# Autodesk Inventor assembly: winch prototype
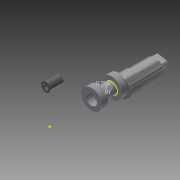
[picture p0: Inventor's stored thumbnail of the model, 180x180]
Saved by Autodesk Inventor 2013 (Build 170138000, 138)
## iProperties
Created: 2013-12-07
Part Number: winch prototype
Document SubType Name: Assembly
Designer: kahohbein
Author: kahohbein
## Documents named in this file (5)
- C:\Users\kahohbein\Documents\GitHub\2013-2014_BlockParty\CAD\Lift\MK2\winch prototype.iam
- C:\Users\kahohbein\Documents\GitHub\2013-2014_BlockParty\CAD\COTSParts\Tetrix\Tetrix hub - motor.ipt
- C:\Users\kahohbein\Documents\GitHub\2013-2014_BlockParty\CAD\COTSParts\Tetrix\Tetrix motor.ipt
- C:\Users\kahohbein\Documents\GitHub\2013-2014_BlockParty\CAD\Lift\MK2\winch pipe.ipt
- C:\Users\kahohbein\Documents\GitHub\2013-2014_BlockParty\CAD\COTSParts\Structural\PVC Spacer 375 Sched 80.ipt
## Components (6 placed, 4 different names)
1. Tetrix motor:1 — Mate:11, Mate:12, Mate:14, Mate:15
2. Tetrix motor:2 — Mate:9, Mate:10, Mate:13
3. Tetrix hub - motor:1 — Mate:11, Mate:12, Mate:16
4. Tetrix hub - motor:2 — Mate:9, Mate:10
5. winch pipe:1 — Mate:15, Mate:16
6. PVC Spacer 375 Sched 80:1
## Relationships (8: Mate 8)
- Mate:9: Tetrix motor:2 ↔ Tetrix hub - motor:2
- Mate:10: Tetrix motor:2 ↔ Tetrix hub - motor:2
- Mate:11: Tetrix motor:1 ↔ Tetrix hub - motor:1
- Mate:12: Tetrix motor:1 ↔ Tetrix hub - motor:1
- Mate:13: Tetrix motor:2
- Mate:14: Tetrix motor:1
- Mate:15: Tetrix motor:1 ↔ winch pipe:1
- Mate:16: Tetrix hub - motor:1 ↔ winch pipe:1
